# Autodesk Inventor assembly: brazo robot
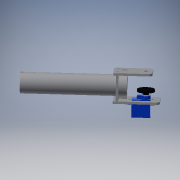
[picture p0: Inventor's stored thumbnail of the model, 180x180]
Saved by Autodesk Inventor 2018 (Build 220112000, 112)
## iProperties
Created: 2020-03-10
Part Number: brazo robot
Material: Genérico
Document SubType Name: Assembly
Designer: sala.ceri
Author: sala.ceri
## Documents named in this file (9)
- C:\Users\david\OneDrive\Documents\robot\ensamble\part8.iam
- C:\Users\david\OneDrive\Documents\robot\piezas\BaseServo.ipt
- C:\Users\david\OneDrive\Documents\robot\tubo.ipt
- C:\Users\david\OneDrive\Documents\robot\tapa.ipt
- C:\Users\david\OneDrive\Documents\robot\piezas\Miniservo.ipt
- C:\Users\david\OneDrive\Documents\robot\muñeca2.ipt
- C:\Users\david\OneDrive\Documents\robot\muñeca3.ipt
- C:\Users\david\OneDrive\Documents\robot\muñeca5.ipt
- C:\Users\david\OneDrive\Documents\robot\muñeca4.ipt
## Components (8 placed, 8 different names)
1. tubo:1 — Coincidencia:63, Coincidencia:64, Nivelación:3, Coincidencia:71, Coincidencia:72, Coincidencia:73
2. tapa:1 — Coincidencia:63, Coincidencia:64, Nivelación:3
3. Miniservo:1 — Coincidencia:77, Coincidencia:78, Coincidencia:83, Coincidencia:84
4. muñeca2:1 — Coincidencia:71, Coincidencia:72, Coincidencia:74, Nivelación:4, Nivelación:5, Coincidencia:76
5. muñeca3:1 — Coincidencia:73, Coincidencia:74, Nivelación:4, Coincidencia:75, Coincidencia:81, Coincidencia:82
6. muñeca5:1 — Nivelación:5, Coincidencia:75, Coincidencia:76, Coincidencia:77, Coincidencia:78
7. muñeca4:1 — Coincidencia:81, Coincidencia:82
8. BaseServo:1 — Coincidencia:83, Coincidencia:84
## Relationships (17: Mate 14, Flush 3)
- Coincidencia:63 [Mate]: tubo:1 ↔ tapa:1
- Coincidencia:64 [Mate]: tubo:1 ↔ tapa:1
- Nivelación:3 [Flush]: tubo:1 ↔ tapa:1
- Coincidencia:71 [Mate]: tubo:1 ↔ muñeca2:1
- Coincidencia:72 [Mate]: tubo:1 ↔ muñeca2:1
- Coincidencia:73 [Mate]: tubo:1 ↔ muñeca3:1
- Coincidencia:74 [Mate]: muñeca2:1 ↔ muñeca3:1
- Nivelación:4 [Flush]: muñeca2:1 ↔ muñeca3:1
- Nivelación:5 [Flush]: muñeca2:1 ↔ muñeca5:1
- Coincidencia:75 [Mate]: muñeca3:1 ↔ muñeca5:1
- Coincidencia:76 [Mate]: muñeca2:1 ↔ muñeca5:1
- Coincidencia:77 [Mate]: Miniservo:1 ↔ muñeca5:1
- Coincidencia:78 [Mate]: Miniservo:1 ↔ muñeca5:1
- Coincidencia:81 [Mate]: muñeca3:1 ↔ muñeca4:1
- Coincidencia:82 [Mate]: muñeca3:1 ↔ muñeca4:1
- Coincidencia:83 [Mate]: Miniservo:1 ↔ BaseServo:1
- Coincidencia:84 [Mate]: Miniservo:1 ↔ BaseServo:1
